# Autodesk Inventor assembly: MZCAT
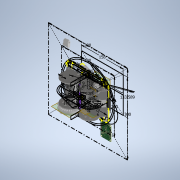
[picture p0: Inventor's stored thumbnail of the model, 180x180]
Saved by Autodesk Inventor 2022 (Build 260153000, 153)
## iProperties
Created: 2024-07-14
Part Number: MZCAT
Document SubType Name: Assembly
Designer: Капустяник Андрей
Author: Капустяник Андрей
## Documents named in this file (42)
- C:\Users\Andrey\Documents\Git\MZCAT_2024\MZCAT.iam
- C:\Users\Andrey\Documents\Git\MZCAT_2024\plan.ipt
- C:\Users\Andrey\Documents\Git\MZCAT_2024\base.ipt
- C:\Users\Andrey\Documents\Git\MZCAT_2024\motor gear.ipt
- C:\Users\Andrey\Documents\Git\MZCAT_2024\motor.ipt
- C:\Users\Andrey\Documents\Git\MZCAT_2024\base plate.ipt
- C:\Users\Andrey\Documents\Git\MZCAT_battery\FastBattery.iam
- C:\Users\Andrey\Documents\Git\MZCAT_2024\akkum_plate.ipt
- C:\Users\Andrey\Documents\Git\MZCAT_2024\CAT_wheel.ipt
- C:\Users\Andrey\Documents\Git\MZCAT_2024\motherCATboard.ipt
- C:\Users\Andrey\Documents\Git\MZCAT_2024\CM4\RaspberryPi_CM4_WithReceptacleH1.5mm.ipt
- C:\Users\Andrey\Documents\Git\MZCAT_2024\labik.ipt
- C:\Users\Andrey\Documents\Git\MZCAT_2024\commutationCATboard.ipt
- C:\Users\Andrey\Documents\Git\MZCAT_2024\LiDAR_LD19_3D_STP_V1.0\LD19.ipt
- C:\Users\Andrey\Documents\Git\MZCAT_2024\CAT_protector.ipt
- C:\Users\Andrey\Documents\Git\MZCAT_2024\MZCAT\Мастер проектирования\Цилиндрическое зубчатое зацепление1.iam
- C:\Users\Andrey\Documents\Git\MZCAT_2024\bearing 37x25x7.ipt
- C:\Users\Andrey\Documents\Git\MZCAT_2024\wheel_shield.ipt
- C:\Users\Andrey\Documents\Git\MZCAT_2024\main_wheel_fixator.ipt
- C:\Users\Andrey\Documents\Git\MZCAT_2024\MZCAT\Мастер проектирования\Цилиндрическое зубчатое зацепление2.iam
- C:\Users\Andrey\Documents\Git\MZCAT_2024\parasit_gear.ipt
- C:\Users\Andrey\Documents\Git\MZCAT_2024\middle_gear_fixator.ipt
- C:\Users\Andrey\Documents\Git\MZCAT_2024\wheel_fixator.ipt
- C:\Users\Andrey\Documents\Git\MZCAT_2024\CAT_slave_wheel.ipt
- C:\Users\Andrey\Documents\Git\MZCAT_2024\wheel_fixator_mirror.ipt
- C:\Users\Andrey\Documents\Git\MZCAT_2024\sensors_frame.ipt
- C:\Users\Andrey\Documents\Git\MZCAT_2024\vydacha_chertezh.ipt
- C:\Users\Andrey\Documents\Git\MZCAT_2024\vydacha_backstenka.ipt
- C:\Users\Andrey\Documents\Git\MZCAT_2024\vzuh_karetka.ipt
- C:\Users\Andrey\Documents\Git\MZCAT_2024\OCS-D008 B.ipt
- C:\Users\Andrey\Documents\Git\MZCAT_2024\magazine.ipt
- C:\Users\Andrey\Documents\Git\MZCAT_2024\28inchdpilcd.ipt
- C:\Users\Andrey\Documents\Git\MZCAT_2024\STL\camera.ipt
- C:\Users\Andrey\Documents\Git\MZCAT_2024\STL\camera fixator.ipt
- C:\Users\Andrey\Documents\Git\MZCAT_2024\Linit Switch.ipt
- C:\Users\Andrey\Documents\Git\MZCAT_2024\push-fit.ipt
- C:\Users\Andrey\Documents\Git\MZCAT_2024\limit_arm.ipt
- C:\Users\Andrey\Documents\Git\MZCAT_2024\vydacha_ServoHolder.ipt
- C:\Users\Andrey\Documents\Git\MZCAT_2024\magazine_fixator.ipt
- C:\Users\Andrey\Documents\Git\MZCAT_2024\shatun_main.ipt
- C:\Users\Andrey\Documents\Git\MZCAT_2024\shatun.ipt
- C:\Users\Andrey\Documents\Git\MZCAT_2024\STL\vydacha planB.ipt
## Components (63 placed, 40 different names)
1. plan:1 — Совмещение:4, Заподлицо:1, Совмещение:5, Совмещение:14, Совмещение:15, Совмещение:20, Совмещение:23, Совмещение:56, Совмещение:60, Совмещение:71, Совмещение:72, Совмещение:73, Совмещение:76
2. base:1 — Совмещение:1, Совмещение:2, Совмещение:3, Совмещение:8, Совмещение:9, Заподлицо:7, Заподлицо:8, Заподлицо:10, Совмещение:17, Заподлицо:11, Заподлицо:13, Совмещение:18, Жесткий:1, Жесткий:2, Совмещение:25, Совмещение:30, Совмещение:35, Заподлицо:94, Заподлицо:95, Заподлицо:102
3. motor gear:1 — Совмещение:6, Заподлицо:3, Совмещение:39, Совмещение:40
4. motor:1 — Совмещение:6, Заподлицо:3, Совмещение:8, Совмещение:10, Заподлицо:10
5. motor gear:2 — Совмещение:7, Заподлицо:2
6. motor:2 — Совмещение:7, Заподлицо:2, Совмещение:9, Совмещение:12, Заподлицо:13
7. base plate:1 — Совмещение:10, Совмещение:17, Заподлицо:11, Совмещение:63, Совмещение:66, Совмещение:67, С поворотом:2, Совмещение:79, Совмещение:80, Совмещение:81, Совмещение:104, Совмещение:112, Заподлицо:95
8. base plate:2 — Совмещение:12, Заподлицо:7, Совмещение:18, Совмещение:52, Совмещение:53, Совмещение:54, Заподлицо:27, Заподлицо:28, Совмещение:103, Совмещение:112, С поворотом:3
9. FastBattery:1 [sub-assembly] — Заподлицо:8, Заподлицо:9, Совмещение:16, Совмещение:28
10. akkum_plate:1 — Жесткий:1
11. CAT_wheel:1 — Совмещение:14, Совмещение:15, Касательность:1, Совмещение:43, Заподлицо:25, Совмещение:44, Совмещение:45, Совмещение:46, Заподлицо:29
12. akkum_plate:2 — Жесткий:2
13. CAT_wheel:3 — Совмещение:20, Совмещение:23, Совмещение:41, Совмещение:42, Заподлицо:26, Заподлицо:30
14. motherCATboard:1 — Совмещение:25, Совмещение:26, Совмещение:30
15. RaspberryPi_CM4_WithReceptacleH1.5mm:1 — Совмещение:31
16. labik:1 — Касательность:1, Заподлицо:17, Совмещение:32, Заподлицо:23, Заподлицо:24
17. commutationCATboard:1 — Совмещение:28, Совмещение:29, Совмещение:31, Совмещение:99, Совмещение:100, Совмещение:121
18. LD19:1 — Заподлицо:16, Совмещение:36, Совмещение:37, Совмещение:113
19. CAT_protector:1 — Совмещение:34, Заподлицо:22, Совмещение:35, Заподлицо:92, Заподлицо:93, Заподлицо:96, Совмещение:114, Совмещение:121
20. Цилиндрическое зубчатое зацепление:1 [sub-assembly] — Совмещение:39, Совмещение:40, Совмещение:41
21. bearing 37x25x7:1 — Совмещение:42, Заподлицо:26, Заподлицо:31
22. bearing 37x25x7:2 — Совмещение:43, Заподлицо:25, Совмещение:47
23. wheel_shield:1 — Совмещение:44, Совмещение:45, Угол:1
24. main_wheel_fixator:1 — Совмещение:46, Совмещение:47, Угол:2
25. Цилиндрическое зубчатое зацепление:2 [sub-assembly] — Совмещение:53, Совмещение:54
26. parasit_gear:1 — Совмещение:52, Совмещение:55
27. middle_gear_fixator:1 — Заподлицо:27, Совмещение:55, С поворотом:3
28. wheel_fixator:1 — Заподлицо:28, Совмещение:56, Угол:3, Совмещение:57, Совмещение:58, Совмещение:68
29. bearing 37x25x7:3 — Совмещение:57, Совмещение:58, Совмещение:59
30. CAT_slave_wheel:1 — Совмещение:59, Заподлицо:29
31. CAT_slave_wheel:2 — Совмещение:60, Заподлицо:30, Совмещение:61
32. bearing 37x25x7:4 — Совмещение:61, Заподлицо:31
33. wheel_fixator_mirror:1 — Совмещение:63, Совмещение:66, Совмещение:67, Совмещение:70
34. wheel_shield:2 — Совмещение:68, Совмещение:71, Угол:6
35. wheel_shield:3 — Совмещение:70, Совмещение:73, Угол:5
36. wheel_shield:4 — Совмещение:72, Угол:4
37. parasit_gear:2 — Совмещение:75, Заподлицо:32
38. middle_gear_fixator:2 — С поворотом:2, Совмещение:75, Заподлицо:32
39. sensors_frame:1 — Совмещение:76, Совмещение:77, Совмещение:78
40. main_wheel_fixator:2 — Совмещение:79, Совмещение:80, Совмещение:81
41. vydacha_chertezh:1 — Совмещение:117, Заподлицо:98, Совмещение:118, Совмещение:123, Совмещение:124, Совмещение:126, Заподлицо:105
42. vydacha_backstenka:1 — Совмещение:116, Совмещение:117, Совмещение:119, Совмещение:120, Совмещение:122
43. vzuh_karetka:1 — Совмещение:119, Совмещение:120, Заподлицо:99, Заподлицо:104
44. OCS-D008 B:1 — Совмещение:124, Совмещение:126, Заподлицо:101, Заподлицо:103, Совмещение:128
45. magazine:1 — Заподлицо:96, Заподлицо:97, Совмещение:114, Совмещение:116, Совмещение:118, Заподлицо:101
46. 28inchdpilcd:1
47. camera:1 — Совмещение:88, Совмещение:91, Совмещение:92
48. camera:2 — Заподлицо:90
49. camera:3 — Совмещение:89
50. camera:4 — Заподлицо:91
51. camera fixator:1 — Совмещение:91, Совмещение:92
52. Linit Switch:1 — Совмещение:93, Совмещение:95, Совмещение:102, Совмещение:104
53. push-fit:1 — Совмещение:94, Совмещение:96, Совмещение:100, Совмещение:101, Заподлицо:92
54. push-fit:2 — Совмещение:93, Совмещение:95, Совмещение:99, Совмещение:102, Заподлицо:93
55. Linit Switch:2 — Совмещение:94, Совмещение:96, Совмещение:101, Совмещение:103
56. limit_arm:1 — Заподлицо:94
57. OCS-D008 B:2 — Совмещение:113
58. OCS-D008 B:3
59. vydacha_ServoHolder:1 — Заподлицо:100, Совмещение:122, Совмещение:123
60. magazine_fixator:1 — Заподлицо:102
61. shatun_main:1 — Заподлицо:103, Совмещение:127, Совмещение:128
62. shatun:1 — Заподлицо:104
63. vydacha planB:1 — Заподлицо:105
## Relationships (142: Mate 93, Flush 38, Angle 6, WeldJoint 2, RevoluteJoint 2, Tangent 1)
- Совмещение:1 [Mate]: base:1
- Совмещение:2 [Mate]: base:1
- Совмещение:3 [Mate]: base:1
- Совмещение:4 [Mate]: plan:1
- Заподлицо:1 [Flush]: plan:1
- Совмещение:5 [Mate]: plan:1
- Совмещение:6 [Mate]: motor gear:1 ↔ motor:1
- Совмещение:7 [Mate]: motor gear:2 ↔ motor:2
- Заподлицо:2 [Flush]: motor gear:2 ↔ motor:2
- Заподлицо:3 [Flush]: motor gear:1 ↔ motor:1
- Совмещение:8 [Mate]: base:1 ↔ motor:1
- Совмещение:9 [Mate]: base:1 ↔ motor:2
- Совмещение:10 [Mate]: motor:1 ↔ base plate:1
- Совмещение:12 [Mate]: motor:2 ↔ base plate:2
- Заподлицо:7 [Flush]: base:1 ↔ base plate:2
- Заподлицо:8 [Flush] (10 mm): base:1 ↔ FastBattery:1
- Заподлицо:9 [Flush]: FastBattery:1
- Совмещение:14 [Mate]: plan:1 ↔ CAT_wheel:1
- Совмещение:15 [Mate]: plan:1 ↔ CAT_wheel:1
- Совмещение:16 [Mate]: FastBattery:1
- Заподлицо:10 [Flush]: base:1 ↔ motor:1
- Совмещение:17 [Mate]: base:1 ↔ base plate:1
- Заподлицо:11 [Flush]: base:1 ↔ base plate:1
- Заподлицо:13 [Flush]: base:1 ↔ motor:2
- Совмещение:18 [Mate]: base:1 ↔ base plate:2
- Жесткий:1 [WeldJoint]: base:1 ↔ akkum_plate:1
- Жесткий:2 [WeldJoint]: base:1 ↔ akkum_plate:2
- Совмещение:20 [Mate]: plan:1 ↔ CAT_wheel:3
- Совмещение:23 [Mate]: plan:1 ↔ CAT_wheel:3
- Совмещение:25 [Mate] (4 mm): base:1 ↔ motherCATboard:1
- Совмещение:26 [Mate]: motherCATboard:1
- Совмещение:28 [Mate] (3 mm): FastBattery:1 ↔ commutationCATboard:1
- Совмещение:29 [Mate]: commutationCATboard:1
- Совмещение:30 [Mate] (1.5 mm): base:1 ↔ motherCATboard:1
- Совмещение:31 [Mate]: RaspberryPi_CM4_WithReceptacleH1.5mm:1 ↔ commutationCATboard:1
- Заподлицо:16 [Flush] (-7.8 mm): LD19:1
- Касательность:1 [Tangent] (3 mm): CAT_wheel:1 ↔ labik:1
- Заподлицо:17 [Flush]: labik:1
- Совмещение:32 [Mate]: labik:1
- Совмещение:34 [Mate]: CAT_protector:1
- Заподлицо:22 [Flush]: CAT_protector:1
- Заподлицо:23 [Flush] (-130 mm): labik:1
- Совмещение:35 [Mate]: base:1 ↔ CAT_protector:1
- Совмещение:36 [Mate]: LD19:1
- Совмещение:37 [Mate]: LD19:1
- Заподлицо:24 [Flush] (-120 mm): labik:1
- Совмещение:39 [Mate]: motor gear:1 ↔ Цилиндрическое зубчатое зацепление:1
- Совмещение:40 [Mate]: motor gear:1 ↔ Цилиндрическое зубчатое зацепление:1
- Совмещение:41 [Mate]: CAT_wheel:3 ↔ Цилиндрическое зубчатое зацепление:1
- Совмещение:42 [Mate]: CAT_wheel:3 ↔ bearing 37x25x7:1
- Совмещение:43 [Mate]: CAT_wheel:1 ↔ bearing 37x25x7:2
- Заподлицо:25 [Flush]: CAT_wheel:1 ↔ bearing 37x25x7:2
- Заподлицо:26 [Flush]: CAT_wheel:3 ↔ bearing 37x25x7:1
- Совмещение:44 [Mate]: CAT_wheel:1 ↔ wheel_shield:1
- Совмещение:45 [Mate] (0.5 mm): CAT_wheel:1 ↔ wheel_shield:1
- Угол:1 [Angle] (180 deg): wheel_shield:1
- Совмещение:46 [Mate] (1 mm): CAT_wheel:1 ↔ main_wheel_fixator:1
- Совмещение:47 [Mate]: bearing 37x25x7:2 ↔ main_wheel_fixator:1
- Угол:2 [Angle] (180 deg): main_wheel_fixator:1
- Совмещение:52 [Mate] (0.25 mm): base plate:2 ↔ parasit_gear:1
- Совмещение:53 [Mate]: base plate:2 ↔ Цилиндрическое зубчатое зацепление:2
- Совмещение:54 [Mate]: base plate:2 ↔ Цилиндрическое зубчатое зацепление:2
- Заподлицо:27 [Flush]: base plate:2 ↔ middle_gear_fixator:1
- Совмещение:55 [Mate]: parasit_gear:1 ↔ middle_gear_fixator:1
- Заподлицо:28 [Flush]: base plate:2 ↔ wheel_fixator:1
- Совмещение:56 [Mate]: plan:1 ↔ wheel_fixator:1
- Угол:3 [Angle] (180 deg): wheel_fixator:1
- Совмещение:57 [Mate]: wheel_fixator:1 ↔ bearing 37x25x7:3
- Совмещение:58 [Mate] (1 mm): wheel_fixator:1 ↔ bearing 37x25x7:3
- Совмещение:59 [Mate]: bearing 37x25x7:3 ↔ CAT_slave_wheel:1
- Заподлицо:29 [Flush]: CAT_wheel:1 ↔ CAT_slave_wheel:1
- Совмещение:60 [Mate]: plan:1 ↔ CAT_slave_wheel:2
- Заподлицо:30 [Flush]: CAT_wheel:3 ↔ CAT_slave_wheel:2
- Совмещение:61 [Mate]: CAT_slave_wheel:2 ↔ bearing 37x25x7:4
- Заподлицо:31 [Flush]: bearing 37x25x7:1 ↔ bearing 37x25x7:4
- Совмещение:63 [Mate]: base plate:1 ↔ wheel_fixator_mirror:1
- Совмещение:66 [Mate]: base plate:1 ↔ wheel_fixator_mirror:1
- Совмещение:67 [Mate]: base plate:1 ↔ wheel_fixator_mirror:1
- Совмещение:68 [Mate] (0.1 mm): wheel_fixator:1 ↔ wheel_shield:2
- Совмещение:70 [Mate] (0.1 mm): wheel_fixator_mirror:1 ↔ wheel_shield:3
- Совмещение:71 [Mate]: plan:1 ↔ wheel_shield:2
- Совмещение:72 [Mate]: plan:1 ↔ wheel_shield:4
- Совмещение:73 [Mate]: plan:1 ↔ wheel_shield:3
- Угол:4 [Angle] (0 deg): wheel_shield:4
- Угол:5 [Angle] (0 deg): wheel_shield:3
- Угол:6 [Angle] (180 deg): wheel_shield:2
- [Mate]: parasit_gear:2 ↔ middle_gear_fixator:2
- С поворотом:2 [RevoluteJoint]: base plate:1 ↔ middle_gear_fixator:2
- Совмещение:75 [Mate]: parasit_gear:2 ↔ middle_gear_fixator:2
- Заподлицо:32 [Flush]: parasit_gear:2 ↔ middle_gear_fixator:2
- Совмещение:76 [Mate]: plan:1 ↔ sensors_frame:1
- Совмещение:77 [Mate]: sensors_frame:1
- Совмещение:78 [Mate]: sensors_frame:1
- Совмещение:79 [Mate]: base plate:1 ↔ main_wheel_fixator:2
- Совмещение:80 [Mate]: base plate:1 ↔ main_wheel_fixator:2
- Совмещение:81 [Mate]: base plate:1 ↔ main_wheel_fixator:2
- Совмещение:88 [Mate]: camera:1
- Заподлицо:90 [Flush]: camera:2
- Совмещение:89 [Mate]: camera:3
- Заподлицо:91 [Flush]: camera:4
- Совмещение:91 [Mate]: camera:1 ↔ camera fixator:1
- Совмещение:92 [Mate] (0.6 mm): camera:1 ↔ camera fixator:1
- Совмещение:93 [Mate] (0.2 mm): Linit Switch:1 ↔ push-fit:2
- Совмещение:94 [Mate] (0.2 mm): push-fit:1 ↔ Linit Switch:2
- Совмещение:95 [Mate] (0.1 mm): Linit Switch:1 ↔ push-fit:2
- Совмещение:96 [Mate] (0.1 mm): push-fit:1 ↔ Linit Switch:2
- Совмещение:99 [Mate]: commutationCATboard:1 ↔ push-fit:2
- Совмещение:100 [Mate]: commutationCATboard:1 ↔ push-fit:1
- Совмещение:101 [Mate]: push-fit:1 ↔ Linit Switch:2
- Заподлицо:92 [Flush] (5 mm): CAT_protector:1 ↔ push-fit:1
- Совмещение:102 [Mate]: Linit Switch:1 ↔ push-fit:2
- Заподлицо:93 [Flush] (5 mm): CAT_protector:1 ↔ push-fit:2
- Совмещение:103 [Mate] (1 mm): base plate:2 ↔ Linit Switch:2
- Совмещение:104 [Mate] (1 mm): base plate:1 ↔ Linit Switch:1
- Заподлицо:94 [Flush]: base:1 ↔ limit_arm:1
- Совмещение:112 [Mate]: base plate:1 ↔ base plate:2
- Заподлицо:95 [Flush]: base:1 ↔ base plate:1
- Совмещение:113 [Mate] (0.5 mm): LD19:1 ↔ OCS-D008 B:2
- Заподлицо:96 [Flush] (0.5 mm): CAT_protector:1 ↔ magazine:1
- Заподлицо:97 [Flush]: magazine:1
- Совмещение:114 [Mate]: CAT_protector:1 ↔ magazine:1
- Совмещение:116 [Mate]: vydacha_backstenka:1 ↔ magazine:1
- Совмещение:117 [Mate]: vydacha_chertezh:1 ↔ vydacha_backstenka:1
- Заподлицо:98 [Flush]: vydacha_chertezh:1
- Совмещение:118 [Mate]: vydacha_chertezh:1 ↔ magazine:1
- Совмещение:119 [Mate] (0.2 mm): vydacha_backstenka:1 ↔ vzuh_karetka:1
- Совмещение:120 [Mate]: vydacha_backstenka:1 ↔ vzuh_karetka:1
- Заподлицо:99 [Flush]: vzuh_karetka:1
- Совмещение:121 [Mate] (5 mm): commutationCATboard:1 ↔ CAT_protector:1
- С поворотом:3 [RevoluteJoint]: base plate:2 ↔ middle_gear_fixator:1
- Заподлицо:100 [Flush]: vydacha_ServoHolder:1
- Совмещение:122 [Mate]: vydacha_backstenka:1 ↔ vydacha_ServoHolder:1
- Совмещение:123 [Mate]: vydacha_chertezh:1 ↔ vydacha_ServoHolder:1
- Совмещение:124 [Mate]: vydacha_chertezh:1 ↔ OCS-D008 B:1
- Совмещение:126 [Mate]: vydacha_chertezh:1 ↔ OCS-D008 B:1
- Заподлицо:101 [Flush] (3 mm): OCS-D008 B:1 ↔ magazine:1
- Заподлицо:102 [Flush]: base:1 ↔ magazine_fixator:1
- Заподлицо:103 [Flush]: OCS-D008 B:1 ↔ shatun_main:1
- Совмещение:127 [Mate]: shatun_main:1
- Совмещение:128 [Mate]: OCS-D008 B:1 ↔ shatun_main:1
- Заподлицо:104 [Flush]: vzuh_karetka:1 ↔ shatun:1
- Заподлицо:105 [Flush]: vydacha_chertezh:1 ↔ vydacha planB:1
## Named parameters: d137_d108 = 0 mm
